# Autodesk Inventor assembly: Final assembly cuz we cool
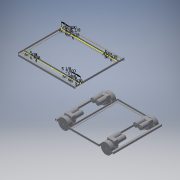
[picture p0: Inventor's stored thumbnail of the model, 180x180]
Saved by Autodesk Inventor 2016 SP2 (Build 200236200, 236)
## iProperties
Created: 2018-01-20
Part Number: Final assembly cuz we cool
Document SubType Name: Assembly
Designer: CAD
Author: CAD
## Documents named in this file (9)
- C:\Users\CAD\Documents\GitHub\FIRST-ROBOTICS-2018-5436-CAD\Robot\Chassis\Final assembly cuz we cool.iam
- C:\Users\CAD\Documents\GitHub\FIRST-ROBOTICS-2018-5436-CAD\Robot\Chassis\27.5 L.ipt
- C:\Users\CAD\Documents\GitHub\FIRST-ROBOTICS-2018-5436-CAD\Robot\Chassis\17.25 L.ipt
- C:\Users\CAD\Documents\GitHub\FIRST-ROBOTICS-2018-5436-CAD\Robot\Chassis\transmission with brackets.iam
- C:\Users\CAD\Documents\GitHub\FIRST-ROBOTICS-2018-5436-CAD\Robot\Chassis\Temp Wheels.ipt
- C:\Users\CAD\Documents\GitHub\FIRST-ROBOTICS-2018-5436-CAD\Robot\Chassis\27 in sq frame.ipt
- C:\Users\CAD\Documents\GitHub\FIRST-ROBOTICS-2018-5436-CAD\Robot\Chassis\32.25 Top L.ipt
- C:\Users\CAD\Documents\GitHub\FIRST-ROBOTICS-2018-5436-CAD\Robot\Chassis\32.25 Top L w holes.ipt
- C:\Users\CAD\Documents\GitHub\FIRST-ROBOTICS-2018-5436-CAD\Robot\Chassis\27.5 Top L.ipt
## Components (20 placed, 8 different names)
1. 27.5 L:1 — Mate:9, Mate:10, Mate:25, Mate:26, Mate:29, Mate:30, Flush:2, Flush:3, Mate:32, Flush:4, Flush:5, Flush:10, Mate:49, Mate:50
2. transmission with brackets:1 [sub-assembly] — Mate:11, Mate:18, Mate:19, Mate:23, Mate:47, Mate:52
3. transmission with brackets:2 [sub-assembly] — Mate:10, Mate:12, Mate:17, Mate:20, Mate:24, Mate:50
4. transmission with brackets:3 [sub-assembly] — Mate:14, Mate:15, Mate:21, Mate:48, Mate:53
5. transmission with brackets:4 [sub-assembly] — Mate:9, Mate:13, Mate:16, Mate:22, Mate:49
6. Temp Wheels:1 — Mate:11, Mate:18, Mate:19, Angle:1
7. Temp Wheels:2 — Mate:13, Mate:16, Mate:22, Angle:3
8. Temp Wheels:3 — Mate:14, Mate:15, Mate:21, Angle:4
9. Temp Wheels:4 — Mate:12, Mate:17, Mate:20, Angle:2
10. 27 in sq frame:1 — Mate:24, Flush:10, Flush:13, Mate:54
11. 27 in sq frame:2 — Mate:23, Flush:9, Flush:12, Flush:13
12. 17.25 L:1 — Mate:29, Mate:30, Flush:2, Mate:31, Flush:5, Mate:33, Flush:6, Angle:3, Angle:4
13. 17.25 L:2 — Mate:25, Mate:26, Flush:3, Mate:32, Flush:4, Flush:9, Mate:55, Angle:1, Angle:2
14. 27.5 L:2 — Mate:31, Mate:33, Flush:6, Mate:47, Mate:48, Flush:12, Mate:52, Mate:53
15. 32.25 Top L:1 — Mate:44, Mate:45, Mate:46
16. 32.25 Top L:2 — Mate:41, Mate:42, Mate:43
17. 32.25 Top L w holes:1 — Mate:36, Mate:37, Mate:38, Mate:39
18. 32.25 Top L w holes:2 — Mate:34, Mate:35, Mate:38, Mate:40, Flush:8
19. 27.5 Top L:1 — Mate:34, Mate:35, Mate:36, Mate:37, Flush:7, Mate:43, Mate:45, Mate:46
20. 27.5 Top L:2 — Mate:39, Flush:7, Mate:40, Flush:8, Mate:41, Mate:42, Mate:44
## Relationships (59: Mate 44, Flush 11, Angle 4)
- Mate:9: 27.5 L:1 ↔ transmission with brackets:4
- Mate:10: 27.5 L:1 ↔ transmission with brackets:2
- Mate:11: transmission with brackets:1 ↔ Temp Wheels:1
- Mate:12: transmission with brackets:2 ↔ Temp Wheels:4
- Mate:13: transmission with brackets:4 ↔ Temp Wheels:2
- Mate:14: transmission with brackets:3 ↔ Temp Wheels:3
- Mate:15: transmission with brackets:3 ↔ Temp Wheels:3
- Mate:16: transmission with brackets:4 ↔ Temp Wheels:2
- Mate:17: transmission with brackets:2 ↔ Temp Wheels:4
- Mate:18: transmission with brackets:1 ↔ Temp Wheels:1
- Mate:19 (9.525 mm): transmission with brackets:1 ↔ Temp Wheels:1
- Mate:20 (9.525 mm): transmission with brackets:2 ↔ Temp Wheels:4
- Mate:21 (9.525 mm): transmission with brackets:3 ↔ Temp Wheels:3
- Mate:22 (9.525 mm): transmission with brackets:4 ↔ Temp Wheels:2
- Mate:23: transmission with brackets:1 ↔ 27 in sq frame:2
- Mate:24: transmission with brackets:2 ↔ 27 in sq frame:1
- Mate:25: 27.5 L:1 ↔ 17.25 L:2
- Mate:26: 27.5 L:1 ↔ 17.25 L:2
- Mate:29: 27.5 L:1 ↔ 17.25 L:1
- Mate:30: 27.5 L:1 ↔ 17.25 L:1
- Flush:2: 27.5 L:1 ↔ 17.25 L:1
- Flush:3: 27.5 L:1 ↔ 17.25 L:2
- Mate:31: 17.25 L:1 ↔ 27.5 L:2
- Mate:32: 27.5 L:1 ↔ 17.25 L:2
- Flush:4: 27.5 L:1 ↔ 17.25 L:2
- Flush:5: 27.5 L:1 ↔ 17.25 L:1
- Mate:33: 17.25 L:1 ↔ 27.5 L:2
- Flush:6: 17.25 L:1 ↔ 27.5 L:2
- Mate:34: 32.25 Top L w holes:2 ↔ 27.5 Top L:1
- Mate:35: 32.25 Top L w holes:2 ↔ 27.5 Top L:1
- Mate:36: 32.25 Top L w holes:1 ↔ 27.5 Top L:1
- Mate:37: 32.25 Top L w holes:1 ↔ 27.5 Top L:1
- Mate:38 (546.1 mm): 32.25 Top L w holes:1 ↔ 32.25 Top L w holes:2
- Mate:39: 32.25 Top L w holes:1 ↔ 27.5 Top L:2
- Flush:7: 27.5 Top L:1 ↔ 27.5 Top L:2
- Mate:40: 32.25 Top L w holes:2 ↔ 27.5 Top L:2
- Flush:8 (76.2 mm): 32.25 Top L w holes:2 ↔ 27.5 Top L:2
- Mate:41: 32.25 Top L:2 ↔ 27.5 Top L:2
- Mate:42: 32.25 Top L:2 ↔ 27.5 Top L:2
- Mate:43: 32.25 Top L:2 ↔ 27.5 Top L:1
- Mate:44: 32.25 Top L:1 ↔ 27.5 Top L:2
- Mate:45: 32.25 Top L:1 ↔ 27.5 Top L:1
- Mate:46: 32.25 Top L:1 ↔ 27.5 Top L:1
- Mate:47: transmission with brackets:1 ↔ 27.5 L:2
- Flush:9: 27 in sq frame:2 ↔ 17.25 L:2
- Flush:10: 27.5 L:1 ↔ 27 in sq frame:1
- Mate:48: transmission with brackets:3 ↔ 27.5 L:2
- Mate:49: 27.5 L:1 ↔ transmission with brackets:4
- Mate:50: 27.5 L:1 ↔ transmission with brackets:2
- Flush:12: 27 in sq frame:2 ↔ 27.5 L:2
- Mate:52: transmission with brackets:1 ↔ 27.5 L:2
- Mate:53: transmission with brackets:3 ↔ 27.5 L:2
- Flush:13: 27 in sq frame:1 ↔ 27 in sq frame:2
- Mate:54: 27 in sq frame:1
- Mate:55: 17.25 L:2
- Angle:1 (0 deg): Temp Wheels:1 ↔ 17.25 L:2
- Angle:2 (0 deg): Temp Wheels:4 ↔ 17.25 L:2
- Angle:3 (0 deg): Temp Wheels:2 ↔ 17.25 L:1
- Angle:4 (0 deg): Temp Wheels:3 ↔ 17.25 L:1
